# Autodesk Inventor assembly: 組合-四人測試版
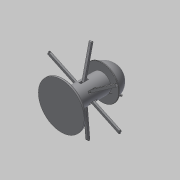
[picture p0: Inventor's stored thumbnail of the model, 180x180]
Saved by Autodesk Inventor 2018 (Build 220112000, 112)
## iProperties
Created: 2021-04-05
Part Number: 組合-四人測試版
Material: 一般
Document SubType Name: Assembly
Designer: 王鼎鈞
Author: 王鼎鈞
## Documents named in this file (6)
- D:\2021顏家民\兩人組圖檔\組合-四人測試版.iam
- D:\2021顏家民\兩人組圖檔\支架3-改良1.ipt
- D:\2021顏家民\兩人組圖檔\支架3-改良1配合.ipt
- D:\2021顏家民\兩人組圖檔\主體.ipt
- D:\2021顏家民\兩人組圖檔\底座構想4.ipt
- D:\2021顏家民\兩人組圖檔\支架3改良組合.iam
## Components (10 placed, 5 different names)
1. 支架3-改良1:1 — 貼合:1, 貼合:2, 插入:2
2. 支架3-改良1配合:1 — 貼合:1, 貼合:2, 相切:1, 相切:2
3. 主體:1 — 插入:1, 插入:2, 插入:3, 插入:4, 插入:5, 插入:6, 插入:7
4. 底座構想4:1 — 插入:1, 相切:1, 相切:2
5. 支架3-改良1配合:2
6. 支架3改良組合:1 [sub-assembly] — 插入:6
7. 支架3改良組合:2 [sub-assembly] — 插入:7
8. 支架3改良組合:3 [sub-assembly] — 插入:5
9. 支架3改良組合:4 [sub-assembly] — 插入:3
10. 支架3改良組合:5 [sub-assembly] — 插入:4
## Relationships (11: Insert 7, Mate 2, Tangent 2)
- 插入:1 [Insert]: 主體:1 ↔ 底座構想4:1
- 貼合:1 [Mate]: 支架3-改良1:1 ↔ 支架3-改良1配合:1
- 貼合:2 [Mate]: 支架3-改良1:1 ↔ 支架3-改良1配合:1
- 插入:2 [Insert]: 支架3-改良1:1 ↔ 主體:1
- 相切:1 [Tangent]: 支架3-改良1配合:1 ↔ 底座構想4:1
- 相切:2 [Tangent]: 支架3-改良1配合:1 ↔ 底座構想4:1
- 插入:3 [Insert]: 主體:1 ↔ 支架3改良組合:4
- 插入:4 [Insert]: 主體:1 ↔ 支架3改良組合:5
- 插入:5 [Insert]: 主體:1 ↔ 支架3改良組合:3
- 插入:6 [Insert]: 主體:1 ↔ 支架3改良組合:1
- 插入:7 [Insert]: 主體:1 ↔ 支架3改良組合:2
